# Autodesk Inventor assembly: Humidifier Assembly
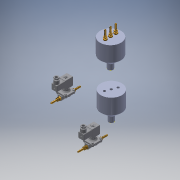
[picture p0: Inventor's stored thumbnail of the model, 180x180]
Saved by Autodesk Inventor 2018 (Build 220112000, 112)
## iProperties
Created: 2020-03-31
Part Number: Humidifier Assembly
Description: STEP AP214
Document SubType Name: Assembly
Designer: emile
Sending System: SolidWorks 2017
Preprocessor: SwSTEP 2.0
Title: Humidifier Assembly.STEP
Revision Number: ANY
## Documents named in this file (4)
- C:\Users\emile\OneDrive\Documents\GitHub\VentilatorCovid19\Respirator\MultiLine\Humidificator\Humidifier Assembly.iam
- C:\Users\emile\OneDrive\Documents\GitHub\VentilatorCovid19\Respirator\MultiLine\Humidificator\Humidifier Botom Funnel.ipt
- C:\Users\emile\OneDrive\Documents\GitHub\VentilatorCovid19\Respirator\MultiLine\SolenoidValve.iam
- C:\Users\emile\OneDrive\Documents\GitHub\VentilatorCovid19\Respirator\Peep\AirPressure\Brass Barbed Hose Fitting for Air and Water.ipt
## Components (7 placed, 4 different names)
1. Humidifier Botom Funnel_1 — Mate:1, Mate:2, Mate:3, Mate:4
2. Humidifier Botom Funnel_2
3. SolenoidValve:1 [sub-assembly]
4. SolenoidValve:2 [sub-assembly]
5. Brass Barbed Hose Fitting for Air and Water:1 — Mate:1, Mate:2, Flush:1
6. Brass Barbed Hose Fitting for Air and Water:2 — Mate:4, Flush:2
7. Brass Barbed Hose Fitting for Air and Water:3 — Mate:3, Flush:1, Flush:2
## Relationships (6: Mate 4, Flush 2)
- Mate:1: Humidifier Botom Funnel_1 ↔ Brass Barbed Hose Fitting for Air and Water:1
- Mate:2: Humidifier Botom Funnel_1 ↔ Brass Barbed Hose Fitting for Air and Water:1
- Mate:3: Humidifier Botom Funnel_1 ↔ Brass Barbed Hose Fitting for Air and Water:3
- Mate:4: Humidifier Botom Funnel_1 ↔ Brass Barbed Hose Fitting for Air and Water:2
- Flush:1: Brass Barbed Hose Fitting for Air and Water:1 ↔ Brass Barbed Hose Fitting for Air and Water:3
- Flush:2: Brass Barbed Hose Fitting for Air and Water:2 ↔ Brass Barbed Hose Fitting for Air and Water:3
